# Autodesk Inventor assembly: ankle_w_feet_left
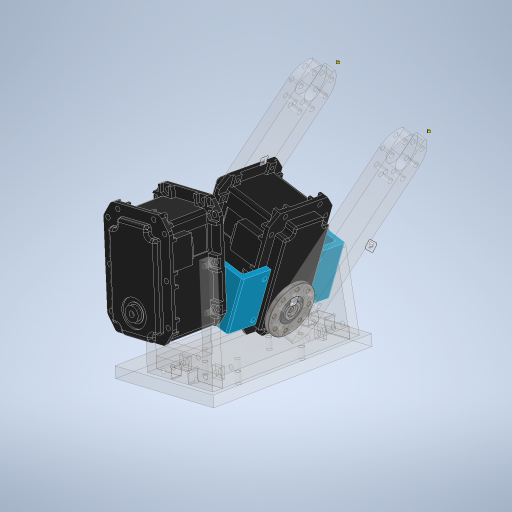
[picture p0: Inventor's stored thumbnail of the model, 512x512]
Saved by Autodesk Inventor 2024 (Build 280153000, 153)
## iProperties
Created: 2024-09-16
Part Number: ankle_w_feet_left
Document SubType Name: Assembly
Designer: jmha0
Author: jmha0
## Documents named in this file (13)
- C:\Users\jmha0\OneDrive\바탕 화면\19th_intern_hjm_fight_robot\부품\Lower_Body\ankle_w_feet\ankle_w_feet_left.iam
- C:\Users\jmha0\OneDrive\바탕 화면\19th_intern_hjm_fight_robot\부품\Lower_Body\feet\feet.ipt
- C:\Users\jmha0\OneDrive\바탕 화면\19th_intern_hjm_fight_robot\부품\Lower_Body\feet\feet_holder1.ipt
- C:\Users\jmha0\OneDrive\바탕 화면\19th_intern_hjm_fight_robot\부품\Lower_Body\feet\feet_holder2.ipt
- C:\Users\jmha0\OneDrive\바탕 화면\19th_intern_hjm_fight_robot\부품\Lower_Body\feet\feet_holder3.ipt
- C:\Users\jmha0\OneDrive\바탕 화면\19th_intern_hjm_fight_robot\부품\hardware\ROBOTIS(Inventor 2024 ver.)\아이들러\64아이들러.iam
- C:\Users\jmha0\OneDrive\바탕 화면\19th_intern_hjm_fight_robot\부품\Lower_Body\ankle_w_motor\3D_ankle1.ipt
- C:\Users\jmha0\OneDrive\바탕 화면\19th_intern_hjm_fight_robot\부품\Lower_Body\ankle_w_motor\3D_ankle2.ipt
- C:\Users\jmha0\OneDrive\바탕 화면\19th_intern_hjm_fight_robot\부품\hardware\ROBOTIS(Inventor 2024 ver.)\혼\64-106Horn.ipt
- C:\Users\jmha0\OneDrive\바탕 화면\19th_intern_hjm_fight_robot\부품\hardware\ROBOTIS(Inventor 2024 ver.)\다이나믹셀\MX-106T+idle.ipt.iam
- C:\Users\jmha0\OneDrive\바탕 화면\19th_intern_hjm_fight_robot\부품\hardware\ROBOTIS(Inventor 2024 ver.)\다이나믹셀\MX-64T.ipt
- C:\Users\jmha0\OneDrive\바탕 화면\19th_intern_hjm_fight_robot\부품\Lower_Body\ankle_w_feet\frame_ankle_to_knee1.ipt
- MX-106T+idle.ipt
## Components (13 placed, 11 different names)
1. feet:1
2. feet_holder1:1 — 삽입:16, 삽입:17, 메이트:1, 각도:1
3. feet_holder2:1 — 삽입:14, 삽입:15, 삽입:25, 삽입:26, 삽입:27
4. feet_holder3:1 — 삽입:14, 삽입:15, 삽입:16, 삽입:17
5. 3D_ankle1:1 — 삽입:18, 삽입:19, 삽입:20, 메이트:2
6. 3D_ankle2:1 — 삽입:21, 삽입:22, 삽입:23
7. 64-106Horn:1 — 메이트:3
8. MX-106T+idle.ipt:1 [sub-assembly] — 삽입:18, 삽입:19, 삽입:20, 삽입:21, 삽입:22, 삽입:23, 메이트:4, 각도:4, 각도:5
9. 64아이들러:1 [sub-assembly] — 메이트:1, 각도:1, 메이트:2
10. MX-64T:1 — 삽입:24, 삽입:25, 삽입:26, 삽입:27
11. 64-106Horn:2 — 삽입:24
12. frame_ankle_to_knee1:1 — 메이트:4, 각도:2, 각도:4, 각도:6, 각도:7
13. frame_ankle_to_knee1:2 — 메이트:3, 각도:2, 각도:5, 각도:6, 각도:7
## Relationships (29: Insert 19, Angle 6, Mate 4)
- [Insert]: feet:1 ↔ feet_holder3:1
- [Insert]: feet:1 ↔ feet_holder3:1
- [Insert]: feet:1 ↔ feet_holder3:1
- [Insert]: feet:1 ↔ feet_holder3:1
- [Insert] (0.1 mm): 64-106Horn:1 ↔ MX-106T+idle.ipt:1
- 삽입:14 [Insert]: feet_holder2:1 ↔ feet_holder3:1
- 삽입:15 [Insert]: feet_holder2:1 ↔ feet_holder3:1
- 삽입:16 [Insert]: feet_holder1:1 ↔ feet_holder3:1
- 삽입:17 [Insert]: feet_holder1:1 ↔ feet_holder3:1
- 메이트:1 [Mate]: feet_holder1:1 ↔ 64아이들러:1
- 각도:1 [Angle] (0 deg): feet_holder1:1 ↔ 64아이들러:1
- 삽입:18 [Insert]: 3D_ankle1:1 ↔ MX-106T+idle.ipt:1
- 삽입:19 [Insert]: 3D_ankle1:1 ↔ MX-106T+idle.ipt:1
- 삽입:20 [Insert]: 3D_ankle1:1 ↔ MX-106T+idle.ipt:1
- 삽입:21 [Insert]: 3D_ankle2:1 ↔ MX-106T+idle.ipt:1
- 삽입:22 [Insert]: 3D_ankle2:1 ↔ MX-106T+idle.ipt:1
- 삽입:23 [Insert]: 3D_ankle2:1 ↔ MX-106T+idle.ipt:1
- 메이트:2 [Mate]: 3D_ankle1:1 ↔ 64아이들러:1
- 삽입:24 [Insert] (0.1 mm): MX-64T:1 ↔ 64-106Horn:2
- 삽입:25 [Insert] (2 mm): feet_holder2:1 ↔ MX-64T:1
- 삽입:26 [Insert] (2 mm): feet_holder2:1 ↔ MX-64T:1
- 삽입:27 [Insert] (2 mm): feet_holder2:1 ↔ MX-64T:1
- 메이트:3 [Mate]: 64-106Horn:1 ↔ frame_ankle_to_knee1:2
- 메이트:4 [Mate]: MX-106T+idle.ipt:1 ↔ frame_ankle_to_knee1:1
- 각도:2 [Angle] (0 deg): frame_ankle_to_knee1:1 ↔ frame_ankle_to_knee1:2
- 각도:4 [Angle] (-30 deg): MX-106T+idle.ipt:1 ↔ frame_ankle_to_knee1:1
- 각도:5 [Angle] (0 deg): MX-106T+idle.ipt:1 ↔ frame_ankle_to_knee1:2
- 각도:6 [Angle] (0 deg): frame_ankle_to_knee1:1 ↔ frame_ankle_to_knee1:2
- 각도:7 [Angle] (0 deg): frame_ankle_to_knee1:1 ↔ frame_ankle_to_knee1:2
## Named parameters: d0_d1 = 0 mm, d1_d2 = 0 mm, d2_d3 = 0 mm
